# Autodesk Inventor assembly: ArkFullTest
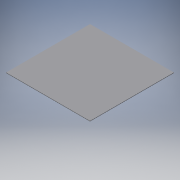
[picture p0: Inventor's stored thumbnail of the model, 180x180]
Saved by Autodesk Inventor 2018 (Build 220112000, 112)
## iProperties
Created: 2019-11-10
Part Number: ArkFullTest
Material: Типовые
Document SubType Name: Assembly
Designer: cosko
Author: cosko
## Documents named in this file (21)
- C:\Users\cosko\source\repos\Arkanoid-robot\Ark.ipt\ArkFullTest.iam
- C:\Users\cosko\source\repos\Arkanoid-robot\Ark.ipt\Up base.ipt
- C:\Users\cosko\source\repos\Arkanoid-robot\Ark.ipt\Motor nema.ipt
- C:\Users\cosko\source\repos\Arkanoid-robot\Ark.ipt\Motor.ipt
- C:\Users\cosko\source\repos\Arkanoid-robot\Ark.ipt\sleeve.ipt
- C:\Users\cosko\source\repos\Arkanoid-robot\Ark.ipt\Wheel.ipt
- C:\Users\cosko\source\repos\Arkanoid-robot\Ark.ipt\Mount for motor.ipt
- C:\Users\cosko\source\repos\Arkanoid-robot\Ark.ipt\FailVersions\Left mount for kick motor.ipt
- C:\Users\cosko\source\repos\Arkanoid-robot\Ark.ipt\FailVersions\Right mount for kick motor.ipt
- C:\Users\cosko\source\repos\Arkanoid-robot\Ark.ipt\FailVersions\Stick.ipt
- C:\Users\cosko\source\repos\Arkanoid-robot\Ark.ipt\Side control right.ipt
- C:\Users\cosko\source\repos\Arkanoid-robot\Ark.ipt\Side control left.ipt
- C:\Users\cosko\source\repos\Arkanoid-robot\Ark.ipt\Down base.ipt
- C:\Users\cosko\source\repos\Arkanoid-robot\Ark.ipt\Screw.ipt
- C:\Users\cosko\source\repos\Arkanoid-robot\Ark.ipt\Shoulder edit .ipt
- C:\Users\cosko\source\repos\Arkanoid-robot\Ather\ipt\Arduino\Arduino Nano.ipt
- C:\Users\cosko\source\repos\Arkanoid-robot\Ark.ipt\Floor.ipt
- C:\Users\cosko\source\repos\Arkanoid-robot\Ark.ipt\Jumper.ipt
- C:\Users\cosko\source\repos\Arkanoid-robot\Ark.ipt\pack for kick motor.ipt
- C:\Users\cosko\source\repos\Arkanoid-robot\Ark.ipt\Kick male.ipt
- C:\Users\cosko\source\repos\Arkanoid-robot\Ark.ipt\Kick female.ipt
## Components (28 placed, 20 different names)
1. Up base:1 — Совмещение:3, Совмещение:4, Совмещение:5, Заподлицо:3, Заподлицо:4, Заподлицо:5, Заподлицо:6, Заподлицо:7, Заподлицо:9, Совмещение:6, Совмещение:7, Совмещение:11, Совмещение:13, Вставка:13, Вставка:14, Вставка:15, Совмещение:14
2. Motor nema:1 — Совмещение:5, Вставка:7, Вставка:8, Вставка:9, Вставка:10, Заподлицо:7, Вставка:21
3. Motor:1 — Совмещение:1, Касательность:1, Вставка:1, Заподлицо:2
4. sleeve:1 — Вставка:1, Вставка:2, Вставка:3
5. Wheel:1 — Вставка:2, Вставка:3, Касательность:3, Заподлицо:8
6. Mount for motor:1 — Совмещение:1, Касательность:1, Совмещение:4, Заподлицо:1, Заподлицо:5
7. Motor:2 — Совмещение:2, Касательность:2, Вставка:4, Заподлицо:2
8. Mount for motor:2 — Совмещение:2, Касательность:2, Совмещение:3, Заподлицо:1, Заподлицо:3, Заподлицо:4, Совмещение:15, Заподлицо:14
9. sleeve:2 — Вставка:4, Вставка:5, Вставка:6
10. Wheel:2 — Вставка:5, Вставка:6, Касательность:4
11. Left mount for kick motor:1 — Вставка:7, Вставка:8
12. Right mount for kick motor:1 — Вставка:9, Вставка:10, Заподлицо:6
13. Stick:1 — Касательность:3, Касательность:4, Заподлицо:8, Заподлицо:9, Совмещение:8, Совмещение:9, Совмещение:10, Совмещение:12, Совмещение:18
14. Side control right:1 — Заподлицо:10, Совмещение:6, Совмещение:7, Совмещение:8, Заподлицо:11
15. Side control left:1 — Заподлицо:10, Совмещение:9, Заподлицо:11
16. Side control right:2 — Заподлицо:12, Заподлицо:13, Совмещение:10, Совмещение:11, Совмещение:13
17. Side control left:2 — Заподлицо:12, Заподлицо:13, Совмещение:12
18. Screw:1 — Вставка:13, Вставка:17
19. Screw:2 — Вставка:14, Вставка:18
20. Screw:3 — Вставка:15, Вставка:16
21. Down base:1 — Вставка:16, Вставка:17, Вставка:18
22. Shoulder edit :1 — Вставка:22, Вставка:23, Вставка:24, Вставка:25
23. Arduino Nano:1 — Совмещение:14, Совмещение:15, Заподлицо:14
24. Floor:1 — Совмещение:18
25. pack for kick motor:1 — Вставка:21, Вставка:22, Вставка:23
26. Jumper:1 — Вставка:24, Вставка:25, Вставка:26, Вставка:27
27. Kick male:1 — Совмещение:19, Совмещение:20, Заподлицо:15, Заподлицо:16, Вставка:26, Вставка:27
28. Kick female:1 — Совмещение:19, Совмещение:20, Заподлицо:15, Заподлицо:16
## Relationships (61: Insert 23, Mate 18, Flush 16, Tangent 4)
- Совмещение:1 [Mate]: Motor:1 ↔ Mount for motor:1
- Касательность:1 [Tangent]: Motor:1 ↔ Mount for motor:1
- Совмещение:2 [Mate]: Motor:2 ↔ Mount for motor:2
- Касательность:2 [Tangent]: Motor:2 ↔ Mount for motor:2
- Вставка:1 [Insert]: Motor:1 ↔ sleeve:1
- Вставка:2 [Insert]: sleeve:1 ↔ Wheel:1
- Вставка:3 [Insert]: sleeve:1 ↔ Wheel:1
- Вставка:4 [Insert]: Motor:2 ↔ sleeve:2
- Вставка:5 [Insert]: sleeve:2 ↔ Wheel:2
- Вставка:6 [Insert]: sleeve:2 ↔ Wheel:2
- Совмещение:3 [Mate]: Up base:1 ↔ Mount for motor:2
- Совмещение:4 [Mate]: Up base:1 ↔ Mount for motor:1
- Совмещение:5 [Mate]: Up base:1 ↔ Motor nema:1
- Заподлицо:1 [Flush]: Mount for motor:1 ↔ Mount for motor:2
- Заподлицо:2 [Flush]: Motor:1 ↔ Motor:2
- Вставка:7 [Insert]: Motor nema:1 ↔ Left mount for kick motor:1
- Вставка:8 [Insert]: Motor nema:1 ↔ Left mount for kick motor:1
- Вставка:9 [Insert]: Motor nema:1 ↔ Right mount for kick motor:1
- Вставка:10 [Insert]: Motor nema:1 ↔ Right mount for kick motor:1
- Заподлицо:3 [Flush] (10 mm): Up base:1 ↔ Mount for motor:2
- Заподлицо:4 [Flush] (20 mm): Up base:1 ↔ Mount for motor:2
- Заподлицо:5 [Flush] (20 mm): Up base:1 ↔ Mount for motor:1
- Заподлицо:6 [Flush] (69.337 mm): Up base:1 ↔ Right mount for kick motor:1
- Заподлицо:7 [Flush] (85.379 mm): Up base:1 ↔ Motor nema:1
- Касательность:3 [Tangent]: Wheel:1 ↔ Stick:1
- Касательность:4 [Tangent]: Wheel:2 ↔ Stick:1
- Заподлицо:8 [Flush] (2.5 mm): Wheel:1 ↔ Stick:1
- Заподлицо:9 [Flush]: Up base:1 ↔ Stick:1
- Заподлицо:10 [Flush]: Side control right:1 ↔ Side control left:1
- Совмещение:6 [Mate]: Up base:1 ↔ Side control right:1
- Совмещение:7 [Mate]: Up base:1 ↔ Side control right:1
- Совмещение:8 [Mate]: Stick:1 ↔ Side control right:1
- Совмещение:9 [Mate]: Stick:1 ↔ Side control left:1
- Заподлицо:11 [Flush]: Side control right:1 ↔ Side control left:1
- Заподлицо:12 [Flush]: Side control right:2 ↔ Side control left:2
- Заподлицо:13 [Flush]: Side control right:2 ↔ Side control left:2
- Совмещение:10 [Mate]: Stick:1 ↔ Side control right:2
- Совмещение:11 [Mate]: Up base:1 ↔ Side control right:2
- Совмещение:12 [Mate]: Stick:1 ↔ Side control left:2
- Совмещение:13 [Mate]: Up base:1 ↔ Side control right:2
- Вставка:13 [Insert]: Up base:1 ↔ Screw:1
- Вставка:14 [Insert]: Up base:1 ↔ Screw:2
- Вставка:15 [Insert]: Up base:1 ↔ Screw:3
- Вставка:16 [Insert]: Screw:3 ↔ Down base:1
- Вставка:17 [Insert]: Screw:1 ↔ Down base:1
- Вставка:18 [Insert]: Screw:2 ↔ Down base:1
- Совмещение:14 [Mate]: Up base:1 ↔ Arduino Nano:1
- Совмещение:15 [Mate]: Mount for motor:2 ↔ Arduino Nano:1
- Заподлицо:14 [Flush]: Mount for motor:2 ↔ Arduino Nano:1
- Совмещение:18 [Mate] (100 mm): Stick:1 ↔ Floor:1
- Вставка:21 [Insert]: Motor nema:1 ↔ pack for kick motor:1
- Вставка:22 [Insert]: Shoulder edit :1 ↔ pack for kick motor:1
- Вставка:23 [Insert]: Shoulder edit :1 ↔ pack for kick motor:1
- Вставка:24 [Insert]: Shoulder edit :1 ↔ Jumper:1
- Вставка:25 [Insert]: Shoulder edit :1 ↔ Jumper:1
- Совмещение:19 [Mate]: Kick male:1 ↔ Kick female:1
- Совмещение:20 [Mate]: Kick male:1 ↔ Kick female:1
- Заподлицо:15 [Flush]: Kick male:1 ↔ Kick female:1
- Заподлицо:16 [Flush]: Kick male:1 ↔ Kick female:1
- Вставка:26 [Insert]: Jumper:1 ↔ Kick male:1
- Вставка:27 [Insert]: Jumper:1 ↔ Kick male:1
